# Autodesk Inventor assembly: Assembly2
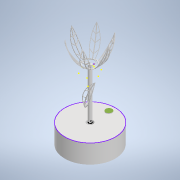
[picture p0: Inventor's stored thumbnail of the model, 180x180]
Saved by Autodesk Inventor 2020.2 (Build 242310000, 310)
## iProperties
Created: 2020-03-02
Part Number: Assembly2
Document SubType Name: Assembly
Designer: lenovo
Author: lenovo
## Documents named in this file (6)
- F:\chinmay\Assembly2.iam
- F:\chinmay\Part2.ipt
- F:\chinmay\Part1.1.ipt
- F:\chinmay\Part3.ipt
- F:\chinmay\Part2.1.ipt
- F:\chinmay\Part2.3.ipt
## Components (10 placed, 5 different names)
1. Part2:1
2. Part1.1:1 — Rotational:1
3. Part3:1 — Rotational:2, Rotational:3, Rotational:4, Rotational:5, Rotational:6, Rotational:7, Rotational:8
4. Part2.1:1 — Rotational:1, Rotational:2
5. Part2.3:1 — Rotational:3
6. Part2.3:2 — Rotational:4
7. Part2.3:3 — Rotational:5
8. Part2.3:4 — Rotational:6
9. Part2.3:5 — Rotational:8
10. Part2.3:6 — Rotational:7
## Relationships (8: RevoluteJoint 8)
- Rotational:1 [RevoluteJoint]: Part1.1:1 ↔ Part2.1:1
- Rotational:2 [RevoluteJoint]: Part3:1 ↔ Part2.1:1
- Rotational:3 [RevoluteJoint]: Part3:1 ↔ Part2.3:1
- Rotational:4 [RevoluteJoint]: Part3:1 ↔ Part2.3:2
- Rotational:5 [RevoluteJoint]: Part3:1 ↔ Part2.3:3
- Rotational:6 [RevoluteJoint]: Part3:1 ↔ Part2.3:4
- Rotational:7 [RevoluteJoint]: Part3:1 ↔ Part2.3:6
- Rotational:8 [RevoluteJoint]: Part3:1 ↔ Part2.3:5
